# Autodesk Inventor assembly: Motor-Wheel Assembly
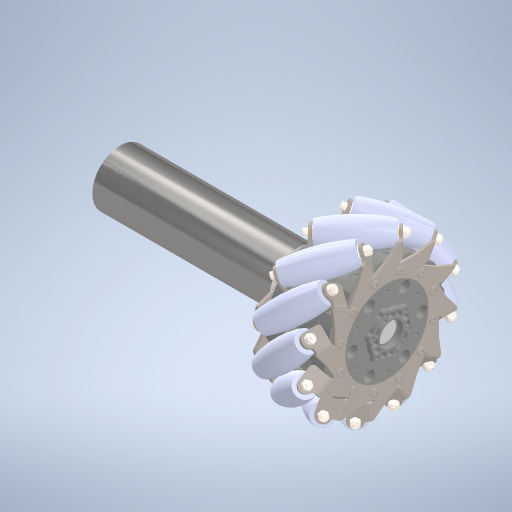
[picture p0: Inventor's stored thumbnail of the model, 512x512]
Saved by Autodesk Inventor 2024 (Build 280153000, 153)
## iProperties
Created: 2023-07-17
Part Number: Motor-Wheel Assembly
Document SubType Name: Assembly
Designer: javie
Author: javie
## Documents named in this file (3)
- C:\Users\javie\OneDrive\Documents\Inventor\L1\WheelSystem.iam
- C:\Users\javie\OneDrive\Documents\Inventor\L1\WheelSystem_Motor.ipt
- C:\Users\javie\OneDrive\Documents\Inventor\L1\WheelSystem_Mecanum.ipt
## Components (2 placed, 2 different names)
1. Motor — Insert:1
2. WheelSystem_Mecanum:1 — Insert:1
## Relationships (1: Insert 1)
- Insert:1: Motor ↔ WheelSystem_Mecanum:1
